# Autodesk Inventor assembly: Sprocket w clamp
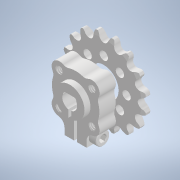
[picture p0: Inventor's stored thumbnail of the model, 180x180]
Saved by Autodesk Inventor 2020 (Build 240168000, 168)
## iProperties
Created: 2020-01-18
Part Number: Sprocket w clamp
Document SubType Name: Assembly
Designer: kevin.nguyen
Author: kevin.nguyen
## Documents named in this file (3)
- C:\Users\tdmp4\OneDrive\Documents\GitHub\CAD-2020\ServoCity\Sprocket w clamp.iam
- C:\Users\tdmp4\OneDrive\Documents\GitHub\CAD-2020\ServoCity\615102.ipt
- C:\Users\tdmp4\OneDrive\Documents\GitHub\CAD-2020\ServoCity\545619 assembly.ipt
## Components (2 placed, 2 different names)
1. 615102:1 — Mate:1, Mate:2, Mate:3
2. 545619 assembly:1 — Mate:1, Mate:2, Mate:3
## Relationships (3: Mate 3)
- Mate:1 (5.08 mm): 615102:1 ↔ 545619 assembly:1
- Mate:2: 615102:1 ↔ 545619 assembly:1
- Mate:3: 615102:1 ↔ 545619 assembly:1
